# Autodesk Inventor assembly: crossAssembly
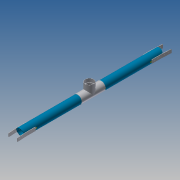
[picture p0: Inventor's stored thumbnail of the model, 180x180]
Saved by Autodesk Inventor 2014 SP1 (Build 180222100, 222)
## iProperties
Created: 2013-12-03
Part Number: crossAssembly
Document SubType Name: Assembly
Designer: Dave
Author: Dave
## Documents named in this file (4)
- C:\Users\Dave\Desktop\hera-cad\surface\crossAssembly.iam
- C:\Users\Dave\Desktop\hera-cad\smallParts\pvc_T_2in.ipt
- C:\Users\Dave\Desktop\hera-cad\surface\cross.ipt
- C:\Users\Dave\Desktop\hera-cad\surface\joinerBracketAB.ipt
## Components (7 placed, 3 different names)
1. pvc_T_2in:1 — Insert:2, Insert:3, Angle:2, Angle:3
2. cross:1 — Insert:2, Angle:3, Insert:5, Angle:5, Insert:6, Angle:6
3. cross:2 — Insert:3, Angle:2, Insert:4, Insert:7, Angle:7, Angle:8
4. joinerBracketAB:1 — Insert:4, Angle:8
5. joinerBracketAB:2 — Insert:5, Angle:5
6. joinerBracketAB:3 — Insert:6, Angle:6
7. joinerBracketAB:4 — Insert:7, Angle:7
## Relationships (12: Insert 6, Angle 6)
- Insert:2 (-24.8 mm): pvc_T_2in:1 ↔ cross:1
- Insert:3 (-24.8 mm): pvc_T_2in:1 ↔ cross:2
- Angle:2 (0 deg): pvc_T_2in:1 ↔ cross:2
- Angle:3 (0 deg): pvc_T_2in:1 ↔ cross:1
- Insert:4: cross:2 ↔ joinerBracketAB:1
- Insert:5: cross:1 ↔ joinerBracketAB:2
- Angle:5 (0 deg): cross:1 ↔ joinerBracketAB:2
- Insert:6: cross:1 ↔ joinerBracketAB:3
- Angle:6 (0 deg): cross:1 ↔ joinerBracketAB:3
- Insert:7: cross:2 ↔ joinerBracketAB:4
- Angle:7 (0 deg): cross:2 ↔ joinerBracketAB:4
- Angle:8 (180 deg): cross:2 ↔ joinerBracketAB:1
## Named parameters: launchAngle = 0 deg
